# Autodesk Inventor assembly: Assembly1
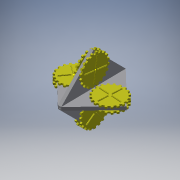
[picture p0: Inventor's stored thumbnail of the model, 180x180]
Saved by Autodesk Inventor 2018.3 (Build 223284000, 284)
## iProperties
Created: 2020-03-24
Part Number: Assembly1
Document SubType Name: Assembly
Designer: ToreDenStore
Author: ToreDenStore
## Documents named in this file (4)
- C:\Users\ToreDenStore\Documents\Inventor\VAWT turbine sunfeather\Assembly1.iam
- C:\Users\ToreDenStore\Documents\Inventor\VAWT turbine sunfeather\MainStructure.ipt
- C:\Users\ToreDenStore\Documents\Inventor\VAWT turbine sunfeather\Double cogwheel.ipt
- C:\Users\ToreDenStore\Documents\Inventor\VAWT turbine sunfeather\Sail.ipt
## Components (7 placed, 3 different names)
1. MainStructure:1 — Insert:1, Insert:2, Insert:3, Insert:4
2. Double cogwheel:1 — Insert:1, Rotation:1
3. Double cogwheel:2 — Insert:2, Rotation:1
4. Double cogwheel:3 — Insert:3, Rotation:2, Rotational:1
5. Double cogwheel:4 — Insert:4, Rotation:2, Rotational:2
6. Sail:1 — Rotational:2
7. Sail:2 — Rotational:1
## Relationships (8: Insert 4, RelateRotation 2, RevoluteJoint 2)
- Insert:1: MainStructure:1 ↔ Double cogwheel:1
- Insert:2: MainStructure:1 ↔ Double cogwheel:2
- Insert:3: MainStructure:1 ↔ Double cogwheel:3
- Insert:4: MainStructure:1 ↔ Double cogwheel:4
- Rotation:1 [RelateRotation] (1 ul): Double cogwheel:1 ↔ Double cogwheel:2
- Rotation:2 [RelateRotation] (-1 ul): Double cogwheel:3 ↔ Double cogwheel:4
- Rotational:1 [RevoluteJoint]: Double cogwheel:3 ↔ Sail:2
- Rotational:2 [RevoluteJoint]: Double cogwheel:4 ↔ Sail:1
